# Autodesk Inventor assembly: RobotAssembly
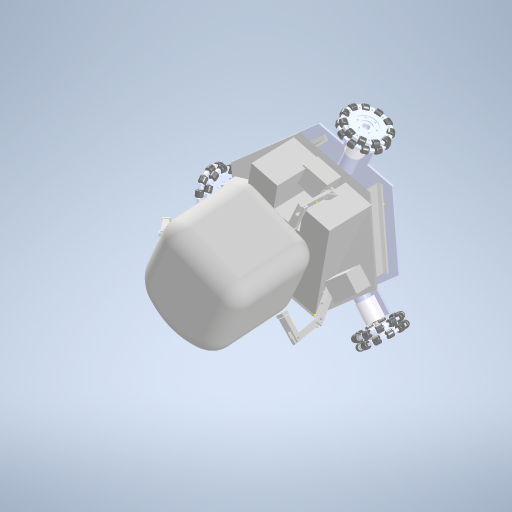
[picture p0: Inventor's stored thumbnail of the model, 512x512]
Saved by Autodesk Inventor 2024 (Build 280153000, 153)
## iProperties
Created: 2023-11-20
Part Number: RobotAssembly
Document SubType Name: Assembly
Designer: prati
Sending System: SolidWorks 2021
Last Author: mrl-iitk
Last Saved: 2023-12-02
Author: prati
## Documents named in this file (7)
- C:\Users\prati\OneDrive - IIT Kanpur\Desktop\Robot\RobotAssembly.iam
- C:\Users\prati\OneDrive - IIT Kanpur\Desktop\Robot\MecanumAssembly.iam
- C:\Users\prati\OneDrive - IIT Kanpur\Desktop\Robot\ArmPlatform.ipt
- C:\Users\prati\OneDrive - IIT Kanpur\Desktop\Robot\ArmMotorSubAssembly.iam
- C:\Users\prati\OneDrive - IIT Kanpur\Desktop\Robot\RobotHeadScaled.ipt
- C:\Users\prati\OneDrive - IIT Kanpur\Desktop\Robot\Tapered.ipt
- C:\Users\prati\OneDrive - IIT Kanpur\Desktop\Robot\ArmMotorSubAssembly_Decoupled.iam
## Components (7 placed, 6 different names)
1. MecanumAssembly:1 [sub-assembly] — Mate:1
2. ArmPlatform:1 — Mate:1, Mate:2, Mate:6, Mate:7, Mate:8, Mate:9, Mate:10
3. ArmMotorSubAssembly:1 [sub-assembly] — Mate:2, Mate:9
4. ArmMotorSubAssembly:3 [sub-assembly] — Mate:8, Mate:10
5. RobotHeadScaled:1
6. Tapered:1 — Mate:7
7. ArmMotorSubAssembly_Decoupled:1 [sub-assembly] — Mate:6
## Relationships (7: Mate 7)
- Mate:1: MecanumAssembly:1 ↔ ArmPlatform:1
- Mate:2: ArmPlatform:1 ↔ ArmMotorSubAssembly:1
- Mate:6: ArmPlatform:1 ↔ ArmMotorSubAssembly_Decoupled:1
- Mate:7: ArmPlatform:1 ↔ Tapered:1
- Mate:8: ArmPlatform:1 ↔ ArmMotorSubAssembly:3
- Mate:9 (10 mm): ArmPlatform:1 ↔ ArmMotorSubAssembly:1
- Mate:10 (50 mm): ArmPlatform:1 ↔ ArmMotorSubAssembly:3
